# Autodesk Inventor assembly: ASY МОО 001 отстойник осветлитель
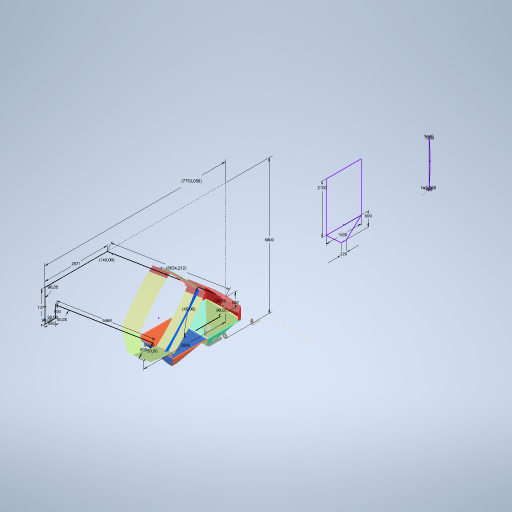
[picture p0: Inventor's stored thumbnail of the model, 512x512]
Saved by Autodesk Inventor 2024.2 (Build 282272000, 272)
## iProperties
Created: 2024-04-28
Part Number: ASY МОО 001 отстойник осветлитель
Document SubType Name: Weldment
Designer: admin
Weld Material: Welded Aluminum-6061
Mass: 420020 g
Surface Area: 719213 cm^2
Volume: 106788 cm^3
Density: 3.93322 g/cm^3
Author: admin
## Documents named in this file (23)
- C:\Users\pokla\Documents\Inventor\Отстойник осветлитель\Manturovo_Se-clar-Gleb\ASY МОО 001 отстойник осветлитель.iam
- C:\Users\pokla\Documents\Inventor\Отстойник осветлитель\Manturovo_Se-clar-Gleb\МОО 020 лист борт 1.ipt
- C:\Users\pokla\Documents\Inventor\Отстойник осветлитель\Manturovo_Se-clar-Gleb\МОО 010 лист спина 1.ipt
- C:\Users\pokla\Documents\Inventor\Отстойник осветлитель\Manturovo_Se-clar-Gleb\Пример емкости.ipt
- C:\Users\pokla\Documents\Inventor\Отстойник осветлитель\Manturovo_Se-clar-Gleb\МОО 030 лист брюхо 1.ipt
- C:\Users\pokla\Documents\Inventor\Отстойник осветлитель\Manturovo_Se-clar-Gleb\МОО 040 шпангоут борт 1.ipt
- C:\Users\pokla\Documents\Inventor\Отстойник осветлитель\Manturovo_Se-clar-Gleb\МОО 041 шпангоут спина 1.ipt
- C:\Users\pokla\Documents\Inventor\Отстойник осветлитель\Manturovo_Se-clar-Gleb\МОО 050 стрингер спина 1.ipt
- C:\Users\pokla\Documents\Inventor\Отстойник осветлитель\Manturovo_Se-clar-Gleb\Рама основания\ASY МОО 040 рама основания.iam
- C:\Users\pokla\Documents\Inventor\Отстойник осветлитель\Manturovo_Se-clar-Gleb\ASY МОО 060 ракета.iam
- C:\Users\pokla\Documents\Inventor\Отстойник осветлитель\Manturovo_Se-clar-Gleb\Content Center Files\en-US\ISO 5251 B 3D\ISO 5251 Bends 3D without straight ends(90 deg) DN80 2 2.ipt
- C:\Users\pokla\Documents\Inventor\Отстойник осветлитель\Manturovo_Se-clar-Gleb\Content Center Files\en-US\ISO 5251(1)\ISO 5251 Concentric reducers DN80 x DN65 3,2 3,2.ipt
- C:\Users\pokla\Documents\Inventor\Отстойник осветлитель\Manturovo_Se-clar-Gleb\ASY МОО 020 конус.iam
- C:\Users\pokla\Documents\Inventor\Отстойник осветлитель\Manturovo_Se-clar-Gleb\ракета\МОО 064 ракета труба.ipt
- C:\Users\pokla\Documents\Inventor\Отстойник осветлитель\Manturovo_Se-clar-Gleb\х_размеры МОО отстойник осветлитель Dummu.ipt
- C:\Users\pokla\Documents\Inventor\Отстойник осветлитель\Manturovo_Se-clar-Gleb\МОО 012 лист спина 2.ipt
- C:\Users\pokla\Documents\Inventor\Отстойник осветлитель\Manturovo_Se-clar-Gleb\ракета\МОО 065 ракета труба 5.ipt
- C:\Users\pokla\Documents\Inventor\Отстойник осветлитель\Manturovo_Se-clar-Gleb\ракета\МОО 066 ракета труба 6.ipt
- C:\Users\pokla\Documents\Inventor\Отстойник осветлитель\Manturovo_Se-clar-Gleb\ракета\МОО 067 ракета труба 7.ipt
- C:\Users\pokla\Documents\Inventor\Отстойник осветлитель\Manturovo_Se-clar-Gleb\Content Center Files\en-US\DIN EN 1092-1 01 - PN 25\DIN EN 1092-1 Plate Flange for Welding Type 01 - PN 25 80 x 88.9.ipt
- C:\Users\pokla\Documents\Inventor\Отстойник осветлитель\Manturovo_Se-clar-Gleb\МОО 011 лист борт.ipt
- C:\Users\pokla\Documents\Inventor\Отстойник осветлитель\Manturovo_Se-clar-Gleb\Листы бака Глеб\МОО 031 Усилитель спина.ipt
- C:\Users\pokla\Documents\Inventor\Отстойник осветлитель\Manturovo_Se-clar-Gleb\Листы бака Глеб\032 Усилитель левый борт.ipt
## Components (36 placed, 22 different names)
1. Пример емкости:1 — Mate:1, Mate:2, Flush:2
2. х_размеры МОО отстойник осветлитель Dummu:1
3. ASY МОО 040 рама основания:1 [sub-assembly] — Flush:19, Flush:20, Flush:21
4. МОО 020 лист борт 1:2 — Angle:1, Symmetry:1
5. МОО 010 лист спина 1:1 — Flush:3, Rigid:11, Rigid:12
6. МОО 020 лист борт 1:1 — Symmetry:1, Flush:8
7. МОО 030 лист брюхо 1:1 — Mate:9, Mate:20, Mate:21, Flush:29
8. МОО 040 шпангоут борт 1:2 — Flush:10, Symmetry:2, Flush:11, Flush:15, Flush:16
9. МОО 041 шпангоут спина 1:2 — Mate:11, Flush:12
10. МОО 040 шпангоут борт 1:1 — Flush:8, Flush:10, Symmetry:2, Flush:11, Mate:11, Flush:14
11. ASY МОО 060 ракета:1 [sub-assembly] — Flush:23, Rigid:10
12. ISO 5251 Bends 3D without straight ends(90 deg) DN80 2:1 — Rigid:2, Rigid:3
13. ISO 5251 Concentric reducers DN80 x DN65 3,2:1 — Rigid:2, Rigid:10
14. ASY МОО 020 конус:1 [sub-assembly] — Flush:22, Mate:16, Flush:28
15. МОО 064 ракета труба:1 — Rigid:3, Cylindrical:1
16. МОО 010 лист спина 1:2 — Rigid:11, Rigid:13, Rigid:14, Rigid:15
17. МОО 010 лист спина 1:3 — Flush:24, Rigid:12, Mate:19
18. МОО 012 лист спина 2:1 — Mate:15, Mate:16, Flush:27, Mate:19
19. МОО 065 ракета труба 5:1 — Rigid:5
20. МОО 066 ракета труба 6:1 — Rigid:5, Rigid:6
21. МОО 067 ракета труба 7:1 — Rigid:6, Rigid:7
22. DIN EN 1092-1 Plate Flange for Welding Type 01 - PN 25 80 x 88.9:1 — Flush:25, Flush:26, Mate:18, Cylindrical:1
23. ISO 5251 Concentric reducers DN80 x DN65 3,2:2 — Rigid:7
24. МОО 010 лист спина 1:4 — Rigid:13
25. МОО 011 лист борт:1 — Rigid:14, Mate:20
26. МОО 011 лист борт:2 — Rigid:15, Mate:21, Flush:29
27. МОО 031 Усилитель спина:1
28. 032 Усилитель левый борт:1
29. МОО 050 стрингер спина 1:1 — Flush:14, Flush:17
30. МОО 050 стрингер спина 1:2 — Flush:15, Flush:16, Flush:17
31. МОО 050 стрингер спина 1:3
32. МОО 050 стрингер спина 1:4
33. МОО 050 стрингер спина 1:5
34. МОО 050 стрингер спина 1:6
35. МОО 050 стрингер спина 1:7
36. МОО 050 стрингер спина 1:8
## Component patterns: (4 elements, first: МОО 050 стрингер спина 1:1 + МОО 050 стрингер спина 1:2)
## Relationships (46: Flush 21, WeldJoint 11, Mate 10, Symmetry 2, Angle 1, CylindricalJoint 1)
- Mate:1: Пример емкости:1
- Mate:2: Пример емкости:1
- Flush:2: Пример емкости:1
- Flush:3: МОО 010 лист спина 1:1
- Angle:1 (180 deg): МОО 020 лист борт 1:2
- Symmetry:1: МОО 020 лист борт 1:2 ↔ МОО 020 лист борт 1:1
- Mate:9: МОО 030 лист брюхо 1:1
- Flush:8: МОО 020 лист борт 1:1 ↔ МОО 040 шпангоут борт 1:1
- Flush:10: МОО 040 шпангоут борт 1:2 ↔ МОО 040 шпангоут борт 1:1
- Symmetry:2: МОО 040 шпангоут борт 1:2 ↔ МОО 040 шпангоут борт 1:1
- Flush:11: МОО 040 шпангоут борт 1:2 ↔ МОО 040 шпангоут борт 1:1
- Mate:11: МОО 041 шпангоут спина 1:2 ↔ МОО 040 шпангоут борт 1:1
- Flush:12: МОО 041 шпангоут спина 1:2
- Flush:14 (3 mm): МОО 040 шпангоут борт 1:1 ↔ МОО 050 стрингер спина 1:1
- Flush:15 (-250 mm): МОО 040 шпангоут борт 1:2 ↔ МОО 050 стрингер спина 1:2
- Flush:16 (3 mm): МОО 040 шпангоут борт 1:2 ↔ МОО 050 стрингер спина 1:2
- Flush:17: МОО 050 стрингер спина 1:1 ↔ МОО 050 стрингер спина 1:2
- Rigid:2 [WeldJoint]: ISO 5251 Bends 3D without straight ends(90 deg) DN80 2:1 ↔ ISO 5251 Concentric reducers DN80 x DN65 3,2:1
- Rigid:3 [WeldJoint]: ISO 5251 Bends 3D without straight ends(90 deg) DN80 2:1 ↔ МОО 064 ракета труба:1
- Flush:19 (-250 mm): ASY МОО 040 рама основания:1
- Flush:20: ASY МОО 040 рама основания:1
- Flush:21: ASY МОО 040 рама основания:1
- Flush:22: ASY МОО 020 конус:1
- Flush:23: ASY МОО 060 ракета:1
- Mate:15: МОО 012 лист спина 2:1
- Flush:24: МОО 010 лист спина 1:3
- Mate:16: ASY МОО 020 конус:1 ↔ МОО 012 лист спина 2:1
- Rigid:5 [WeldJoint]: МОО 065 ракета труба 5:1 ↔ МОО 066 ракета труба 6:1
- Rigid:6 [WeldJoint]: МОО 066 ракета труба 6:1 ↔ МОО 067 ракета труба 7:1
- Flush:25: DIN EN 1092-1 Plate Flange for Welding Type 01 - PN 25 80 x 88.9:1
- Flush:26: DIN EN 1092-1 Plate Flange for Welding Type 01 - PN 25 80 x 88.9:1
- Mate:18 (120 mm): DIN EN 1092-1 Plate Flange for Welding Type 01 - PN 25 80 x 88.9:1
- Rigid:7 [WeldJoint]: МОО 067 ракета труба 7:1 ↔ ISO 5251 Concentric reducers DN80 x DN65 3,2:2
- Rigid:10 [WeldJoint] (-20 mm): ASY МОО 060 ракета:1 ↔ ISO 5251 Concentric reducers DN80 x DN65 3,2:1
- Cylindrical:1: МОО 064 ракета труба:1 ↔ DIN EN 1092-1 Plate Flange for Welding Type 01 - PN 25 80 x 88.9:1
- Flush:27 (40 mm): МОО 012 лист спина 2:1
- Flush:28: ASY МОО 020 конус:1
- Rigid:11 [WeldJoint]: МОО 010 лист спина 1:1 ↔ МОО 010 лист спина 1:2
- Rigid:12 [WeldJoint]: МОО 010 лист спина 1:1 ↔ МОО 010 лист спина 1:3
- Mate:19: МОО 010 лист спина 1:3 ↔ МОО 012 лист спина 2:1
- Rigid:13 [WeldJoint]: МОО 010 лист спина 1:2 ↔ МОО 010 лист спина 1:4
- Rigid:14 [WeldJoint] (-25 mm): МОО 010 лист спина 1:2 ↔ МОО 011 лист борт:1
- Rigid:15 [WeldJoint] (-25 mm): МОО 010 лист спина 1:2 ↔ МОО 011 лист борт:2
- Mate:20: МОО 030 лист брюхо 1:1 ↔ МОО 011 лист борт:1
- Mate:21: МОО 030 лист брюхо 1:1 ↔ МОО 011 лист борт:2
- Flush:29: МОО 030 лист брюхо 1:1 ↔ МОО 011 лист борт:2
## Named parameters: Бак_нахлест_фланца = 25 mm
